# Autodesk Inventor assembly: Upper Stage
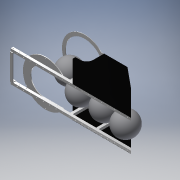
[picture p0: Inventor's stored thumbnail of the model, 180x180]
Saved by Autodesk Inventor 2019.4 (Build 234330000, 330)
## iProperties
Created: 2020-01-18
Part Number: Upper Stage
Document SubType Name: Assembly
Designer: Mark
Mass: 3221.01 g
Surface Area: 17103.2 cm^2
Volume: 13017 cm^3
Density: 0.247448 g/cm^3
Author: Mark
## Documents named in this file (14)
- C:\Users\admin\Desktop\FRC 2020 Engineering\GitHub\7738-2020\Upper Stage\Upper Stage.iam
- C:\Users\admin\Desktop\FRC 2020 Engineering\GitHub\7738-2020\Upper Stage\Main Extrusions.ipt
- C:\Users\admin\Desktop\FRC 2020 Engineering\GitHub\7738-2020\Upper Stage\Back Support Piece.ipt
- C:\Users\admin\Desktop\FRC 2020 Engineering\GitHub\7738-2020\Upper Stage\Secondary Extrusions.ipt
- C:\Users\admin\Desktop\FRC 2020 Engineering\GitHub\7738-2020\Power Cell.ipt
- C:\Users\admin\Desktop\FRC 2020 Engineering\GitHub\7738-2020\Upper Stage\First stage shaft.ipt
- C:\Users\admin\Desktop\FRC 2020 Engineering\GitHub\7738-2020\Upper Stage\KFL08.ipt
- C:\Users\admin\Desktop\FRC 2020 Engineering\GitHub\7738-2020\Upper Stage\Turret Support.ipt
- C:\Users\admin\Desktop\FRC 2020 Engineering\GitHub\7738-2020\Upper Stage\HTD 5M 15 Teeth.ipt
- C:\Users\admin\Desktop\FRC 2020 Engineering\GitHub\7738-2020\Upper Stage\HTD 5M 775.ipt
- C:\Users\admin\Desktop\FRC 2020 Engineering\GitHub\7738-2020\Upper Stage\Turret Support 2.ipt
- C:\Users\admin\Desktop\FRC 2020 Engineering\GitHub\7738-2020\Upper Stage\Side Plates.ipt
- C:\Users\admin\Desktop\FRC 2020 Engineering\GitHub\7738-2020\Upper Stage\Vertical Support 1.ipt
- C:\Users\admin\Desktop\FRC 2020 Engineering\GitHub\7738-2020\Upper Stage\Vertical Support 2.ipt
## Components (30 placed, 13 different names)
1. Main Extrusions:1 — Mate:1, Flush:1, Flush:2, Flush:8, Flush:11, Mate:20, Mate:21
2. Main Extrusions:2 — Mate:1, Flush:1, Flush:2, Flush:3, Flush:4, Mate:2, Flush:5, Flush:7, Mate:3, Flush:20, Mate:31, Flush:21
3. Back Support Piece:1 — Flush:3, Flush:4, Mate:2
4. Secondary Extrusions:1 — Flush:5, Flush:7, Flush:9, Mate:3, Mate:4, Mate:5, Mate:6, Mate:13, Mate:14, Mate:15, Flush:15, Mate:30, Flush:18, Flush:19
5. Secondary Extrusions:2 — Flush:8, Flush:9, Mate:7, Mate:8, Mate:9, Mate:10, Mate:11, Mate:12, Flush:14, Flush:15, Flush:16, Flush:17, Mate:29
6. Power Cell:1
7. Power Cell:2
8. Power Cell:3
9. Power Cell:4
10. First stage shaft:1 — Mate:16, Mate:17, Mate:22, Flush:12
11. KFL08:1 — Mate:4, Mate:5, Mate:6
12. KFL08:2 — Mate:7, Mate:8, Mate:9, Mate:16, Mate:17
13. KFL08:3 — Mate:13, Mate:14, Mate:15
14. KFL08:4 — Mate:10, Mate:11, Mate:12, Mate:18, Mate:19
15. First stage shaft:2 — Mate:18, Mate:19, Mate:23, Flush:13
16. Turret Support:1 — Flush:11, Mate:20, Mate:21, Mate:27, Mate:28
17. HTD 5M 15 Teeth:1 — Mate:22, Flush:12, Mate:24
18. HTD 5M 15 Teeth:2 — Mate:23, Flush:13, Mate:25, Mate:26
19. HTD 5M 775:1 — Mate:24, Mate:25, Mate:26
20. Turret Support 2:1 — Mate:27, Mate:28, Flush:14, Mate:35, Flush:28, Flush:29, Flush:30, Mate:36, Flush:31, Mate:37, Mate:39
21. Side Plates:1 — Flush:16, Flush:17, Mate:29
22. Side Plates:2 — Mate:30, Flush:18, Flush:19
23. Vertical Support 1:1 — Flush:20, Mate:31, Flush:21, Flush:22, Flush:23, Mate:32
24. Vertical Support 1:2 — Flush:22, Flush:23, Mate:32, Flush:26, Mate:34, Flush:27
25. Vertical Support 1:3
26. Vertical Support 1:4 — Flush:26, Mate:34, Flush:27
27. Vertical Support 2:1 — Mate:35, Flush:28, Flush:29, Flush:33, Mate:40
28. Vertical Support 2:2 — Flush:30, Mate:36, Flush:31, Flush:32, Mate:38
29. Vertical Support 2:3 — Flush:33, Mate:39, Mate:40
30. Vertical Support 2:4 — Flush:32, Mate:37, Mate:38
## Relationships (71: Mate 40, Flush 31)
- Mate:1 (200 mm): Main Extrusions:1 ↔ Main Extrusions:2
- Flush:1: Main Extrusions:1 ↔ Main Extrusions:2
- Flush:2: Main Extrusions:1 ↔ Main Extrusions:2
- Flush:3: Main Extrusions:2 ↔ Back Support Piece:1
- Flush:4: Main Extrusions:2 ↔ Back Support Piece:1
- Mate:2: Main Extrusions:2 ↔ Back Support Piece:1
- Flush:5: Main Extrusions:2 ↔ Secondary Extrusions:1
- Flush:7: Main Extrusions:2 ↔ Secondary Extrusions:1
- Flush:8: Main Extrusions:1 ↔ Secondary Extrusions:2
- Flush:9: Secondary Extrusions:1 ↔ Secondary Extrusions:2
- Mate:3 (150 mm): Main Extrusions:2 ↔ Secondary Extrusions:1
- Mate:4: Secondary Extrusions:1 ↔ KFL08:1
- Mate:5: Secondary Extrusions:1 ↔ KFL08:1
- Mate:6: Secondary Extrusions:1 ↔ KFL08:1
- Mate:7: Secondary Extrusions:2 ↔ KFL08:2
- Mate:8: Secondary Extrusions:2 ↔ KFL08:2
- Mate:9: Secondary Extrusions:2 ↔ KFL08:2
- Mate:10: Secondary Extrusions:2 ↔ KFL08:4
- Mate:11: Secondary Extrusions:2 ↔ KFL08:4
- Mate:12: Secondary Extrusions:2 ↔ KFL08:4
- Mate:13: Secondary Extrusions:1 ↔ KFL08:3
- Mate:14: Secondary Extrusions:1 ↔ KFL08:3
- Mate:15: Secondary Extrusions:1 ↔ KFL08:3
- Mate:16: First stage shaft:1 ↔ KFL08:2
- Mate:17 (0.2 mm): First stage shaft:1 ↔ KFL08:2
- Mate:18: KFL08:4 ↔ First stage shaft:2
- Mate:19 (0.2 mm): KFL08:4 ↔ First stage shaft:2
- Flush:11: Main Extrusions:1 ↔ Turret Support:1
- Mate:20: Main Extrusions:1 ↔ Turret Support:1
- Mate:21: Main Extrusions:1 ↔ Turret Support:1
- Mate:22: First stage shaft:1 ↔ HTD 5M 15 Teeth:1
- Flush:12 (-10.5 mm): First stage shaft:1 ↔ HTD 5M 15 Teeth:1
- Mate:23: First stage shaft:2 ↔ HTD 5M 15 Teeth:2
- Flush:13 (-10.5 mm): First stage shaft:2 ↔ HTD 5M 15 Teeth:2
- Mate:24: HTD 5M 15 Teeth:1 ↔ HTD 5M 775:1
- Mate:25: HTD 5M 15 Teeth:2 ↔ HTD 5M 775:1
- Mate:26 (0.5 mm): HTD 5M 15 Teeth:2 ↔ HTD 5M 775:1
- Mate:27 (296.424 mm): Turret Support:1 ↔ Turret Support 2:1
- Mate:28: Turret Support:1 ↔ Turret Support 2:1
- Flush:14: Secondary Extrusions:2 ↔ Turret Support 2:1
- Flush:15: Secondary Extrusions:1 ↔ Secondary Extrusions:2
- Flush:16: Secondary Extrusions:2 ↔ Side Plates:1
- Flush:17: Secondary Extrusions:2 ↔ Side Plates:1
- Mate:29: Secondary Extrusions:2 ↔ Side Plates:1
- Mate:30: Secondary Extrusions:1 ↔ Side Plates:2
- Flush:18: Secondary Extrusions:1 ↔ Side Plates:2
- Flush:19: Secondary Extrusions:1 ↔ Side Plates:2
- Flush:20: Main Extrusions:2 ↔ Vertical Support 1:1
- Mate:31: Main Extrusions:2 ↔ Vertical Support 1:1
- Flush:21 (640 mm): Main Extrusions:2 ↔ Vertical Support 1:1
- Flush:22: Vertical Support 1:1 ↔ Vertical Support 1:2
- Flush:23: Vertical Support 1:1 ↔ Vertical Support 1:2
- Mate:32 (180 mm): Vertical Support 1:1 ↔ Vertical Support 1:2
- [Flush]: Vertical Support 1:3 ↔ Vertical Support 1:4
- [Flush]: Vertical Support 1:3 ↔ Vertical Support 1:4
- [Mate] (180 mm): Vertical Support 1:3 ↔ Vertical Support 1:4
- Flush:26: Vertical Support 1:2 ↔ Vertical Support 1:4
- Mate:34 (200 mm): Vertical Support 1:2 ↔ Vertical Support 1:4
- Flush:27: Vertical Support 1:2 ↔ Vertical Support 1:4
- Mate:35: Turret Support 2:1 ↔ Vertical Support 2:1
- Flush:28: Turret Support 2:1 ↔ Vertical Support 2:1
- Flush:29: Turret Support 2:1 ↔ Vertical Support 2:1
- Flush:30: Turret Support 2:1 ↔ Vertical Support 2:2
- Mate:36: Turret Support 2:1 ↔ Vertical Support 2:2
- Flush:31: Turret Support 2:1 ↔ Vertical Support 2:2
- Flush:32: Vertical Support 2:2 ↔ Vertical Support 2:4
- Mate:37: Turret Support 2:1 ↔ Vertical Support 2:4
- Mate:38 (140 mm): Vertical Support 2:2 ↔ Vertical Support 2:4
- Flush:33: Vertical Support 2:1 ↔ Vertical Support 2:3
- Mate:39: Turret Support 2:1 ↔ Vertical Support 2:3
- Mate:40 (140 mm): Vertical Support 2:1 ↔ Vertical Support 2:3
## Named parameters: d56_d53 = 0 mm, d57_d54 = 0 mm, d58_d55 = 180 mm
